# Autodesk Inventor assembly: trumpet pieces assembly
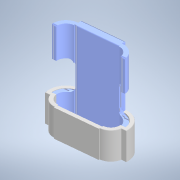
[picture p0: Inventor's stored thumbnail of the model, 180x180]
Saved by Autodesk Inventor 2020 (Build 240168000, 168)
## iProperties
Created: 2020-02-09
Part Number: trumpet pieces assembly
Document SubType Name: Assembly
Designer: Ball
Author: Ball
## Documents named in this file (4)
- C:\TrumpetAdaptiveDevice\trumpet pieces assembly.iam
- C:\TrumpetAdaptiveDevice\Valves.ipt
- C:\TrumpetAdaptiveDevice\Real bottom.ipt
- C:\TrumpetAdaptiveDevice\valve holder.ipt
## Components (3 placed, 3 different names)
1. Valves:1 — Mate:1, Mate:2, Mate:3, Mate:4, Mate:5
2. Real bottom:1 — Mate:1, Mate:2, Mate:3, Flush:1
3. valve holder:1 — Mate:4, Mate:5, Flush:1
## Relationships (6: Mate 5, Flush 1)
- Mate:1: Valves:1 ↔ Real bottom:1
- Mate:2: Valves:1 ↔ Real bottom:1
- Mate:3: Valves:1 ↔ Real bottom:1
- Mate:4: Valves:1 ↔ valve holder:1
- Mate:5: Valves:1 ↔ valve holder:1
- Flush:1: Real bottom:1 ↔ valve holder:1
